# Autodesk Inventor assembly: Assembly
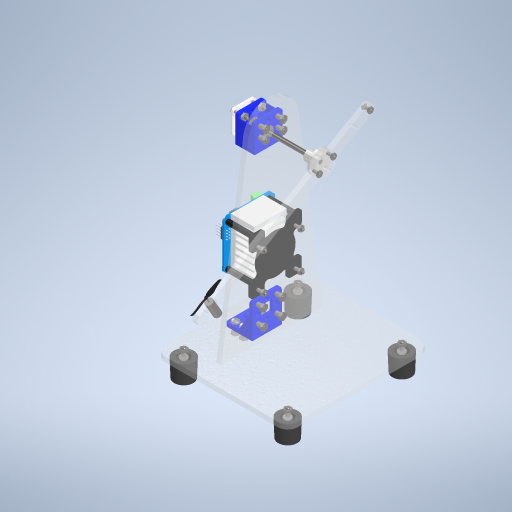
[picture p0: Inventor's stored thumbnail of the model, 512x512]
Saved by Autodesk Inventor 2023.1 (Build 271208000, 208)
## iProperties
Created: 2023-05-07
Part Number: Assembly
Document SubType Name: Assembly
Designer: felip
Author: felip
## Documents named in this file (25)
- C:\Users\felip\OneDrive\UNAL FORE\SEMESTRE 9\TECNICAS DE CONTROL\PROYECTO\PROYECTO-TDC-INVENTOR\Assembly.iam
- C:\Users\felip\OneDrive\UNAL FORE\SEMESTRE 9\TECNICAS DE CONTROL\PROYECTO\PROYECTO-TDC-INVENTOR\base.ipt
- C:\Users\felip\OneDrive\UNAL FORE\SEMESTRE 9\TECNICAS DE CONTROL\PROYECTO\PROYECTO-TDC-INVENTOR\Pata-Goma.ipt
- C:\Users\felip\OneDrive\UNAL FORE\SEMESTRE 9\TECNICAS DE CONTROL\PROYECTO\PROYECTO-TDC-INVENTOR\BaseParal.ipt
- C:\Users\felip\OneDrive\UNAL FORE\SEMESTRE 9\TECNICAS DE CONTROL\PROYECTO\PROYECTO-TDC-INVENTOR\SoporteUnion.ipt
- C:\Users\felip\OneDrive\UNAL FORE\SEMESTRE 9\TECNICAS DE CONTROL\PROYECTO\PROYECTO-TDC-INVENTOR\SoporteEncoder.ipt
- C:\Users\felip\OneDrive\UNAL FORE\SEMESTRE 9\TECNICAS DE CONTROL\PROYECTO\PROYECTO-TDC-INVENTOR\rodamiento.ipt
- C:\Users\felip\OneDrive\UNAL FORE\SEMESTRE 9\TECNICAS DE CONTROL\PROYECTO\PROYECTO-TDC-INVENTOR\topito.ipt
- C:\Users\felip\OneDrive\UNAL FORE\SEMESTRE 9\TECNICAS DE CONTROL\PROYECTO\PROYECTO-TDC-INVENTOR\brida.ipt
- C:\Users\felip\OneDrive\UNAL FORE\SEMESTRE 9\TECNICAS DE CONTROL\PROYECTO\PROYECTO-TDC-INVENTOR\eje.ipt
- C:\Users\felip\OneDrive\UNAL FORE\SEMESTRE 9\TECNICAS DE CONTROL\PROYECTO\PROYECTO-TDC-INVENTOR\brazo.ipt
- C:\Users\felip\OneDrive\UNAL FORE\SEMESTRE 9\TECNICAS DE CONTROL\PROYECTO\PROYECTO-TDC-INVENTOR\motor.ipt
- C:\Users\felip\OneDrive\UNAL FORE\SEMESTRE 9\TECNICAS DE CONTROL\PROYECTO\PROYECTO-TDC-INVENTOR\helice.ipt
- C:\Users\felip\OneDrive\UNAL FORE\SEMESTRE 9\TECNICAS DE CONTROL\PROYECTO\PROYECTO-TDC-INVENTOR\AS5600 v1.ipt
- C:\Users\felip\OneDrive\Documents\Inventor\Content Center Files\R2023\en-US\BS 4183(7)\BS 4183 - M3,5 x 8(2) III.ipt
- C:\Users\felip\OneDrive\Documents\Inventor\Content Center Files\R2023\en-US\BS 4183(4)\BS 4183 - M3,5 x 10(1) III.ipt
- C:\Users\felip\OneDrive\Documents\Inventor\Content Center Files\R2023\en-US\BS 4183(4)\BS 4183 - M2,5 x 10(1) III.ipt
- C:\Users\felip\OneDrive\Documents\Inventor\Content Center Files\R2023\en-US\BS 4183(4)\BS 4183 - M2,5 x 14(1) III.ipt
- C:\Users\felip\OneDrive\Documents\Inventor\Content Center Files\R2023\en-US\BS 4183(4)\BS 4183 - M2,5 x 9(1) III.ipt
- C:\Users\felip\OneDrive\Documents\Inventor\Content Center Files\R2023\en-US\BS 4183(4)\BS 4183 - M2,5 x 7(1) III.ipt
- C:\Users\felip\OneDrive\Documents\Inventor\Content Center Files\R2023\en-US\BS 4183(1)\BS 4183 - M3,5(1).ipt
- C:\Users\felip\OneDrive\Documents\Inventor\Content Center Files\R2023\en-US\BS 4183(1)\BS 4183 - M2,5(1).ipt
- C:\Users\felip\OneDrive\UNAL FORE\SEMESTRE 9\TECNICAS DE CONTROL\PROYECTO\PROYECTO-TDC-INVENTOR\BTS7960 43A HIGH POWER H BRIDGE MODULE.iam
- C:\Users\felip\OneDrive\UNAL FORE\SEMESTRE 9\TECNICAS DE CONTROL\PROYECTO\PROYECTO-TDC-INVENTOR\soporteHBridge.ipt
- C:\Users\felip\OneDrive\Documents\Inventor\Content Center Files\R2023\en-US\BS 4183(4)\BS 4183 - M3 x 7(1) III.ipt
## Components (74 placed, 24 different names)
1. base:1 — Rotational:1, Rotational:2, Rotational:3, Rotational:4, Mate:1, Mate:2, Rotational:5, Rotational:6, Insert:4, Insert:5, Insert:6, Insert:7, Insert:39, Insert:44, Insert:45, Insert:46, Insert:60, Insert:61, Insert:62, Insert:63
2. Pata-Goma:1 — Rotational:1
3. Pata-Goma:2 — Rotational:2
4. Pata-Goma:3 — Rotational:3
5. Pata-Goma:4 — Rotational:4
6. BaseParal:1 — Mate:1, Mate:3, Rotational:7, Rotational:10, Rotational:11, Insert:47, Insert:48, Insert:49, Insert:50, Insert:51, Insert:53, Insert:54, Insert:55, Insert:56, Insert:57, Insert:58, Insert:59, Mate:8, Rotational:20, Rotational:21
7. SoporteUnion:1 — Mate:2, Rotational:5, Rotational:6, Mate:3, Rotational:7, Insert:8, Insert:10, Insert:11, Insert:12, Insert:13, Insert:15, Insert:17, Insert:18
8. SoporteEncoder:1 — Rotational:10, Rotational:11, Insert:1, Insert:2, Rotational:12, Rotational:13, Insert:29, Insert:30, Insert:31, Insert:33, Insert:67, Insert:68
9. rodamiento:1 — Insert:2, Rotational:14
10. rodamiento:2 — Insert:1
11. topito:1 — Rotational:12, Rotational:18
12. topito:2 — Rotational:13, Rotational:19
13. brida:1 — Insert:3, Mate:6, Rotational:15, Rotational:16, Insert:34, Insert:36
14. eje:1 — Rotational:14, Insert:3
15. brazo:1 — Mate:6, Rotational:15, Rotational:16, Flush:1, Tangent:1, Tangent:2, Insert:38, Insert:64, Insert:65, Insert:66
16. motor:1 — Flush:1, Tangent:1, Angle:1, Mate:7, Rotational:17
17. helice:1 — Rotational:17
18. AS5600 v1:1 — Rotational:18, Rotational:19, Insert:25, Insert:28
19. BS 4183 Slotted Pan Head Machine Screw - Metric M3,5 x 8:1 — Insert:4
20. BS 4183 Slotted Pan Head Machine Screw - Metric M3,5 x 8:2 — Insert:5
21. BS 4183 Slotted Pan Head Machine Screw - Metric M3,5 x 8:3 — Insert:6
22. BS 4183 Slotted Pan Head Machine Screw - Metric M3,5 x 8:4 — Insert:7
23. BS 4183 Specification for machine screws and machine screw nuts. Metric series - Metric M3,5 x 10:1 — Insert:8
24. BS 4183 Specification for machine screws and machine screw nuts. Metric series - Metric M3,5 x 10:3 — Insert:10
25. BS 4183 Specification for machine screws and machine screw nuts. Metric series - Metric M3,5 x 10:4 — Insert:11
26. BS 4183 Specification for machine screws and machine screw nuts. Metric series - Metric M3,5 x 10:5 — Insert:12
27. BS 4183 Specification for machine screws and machine screw nuts. Metric series - Metric M3,5 x 10:6 — Insert:13
28. BS 4183 Specification for machine screws and machine screw nuts. Metric series - Metric M3,5 x 10:8 — Insert:15
29. BS 4183 Specification for machine screws and machine screw nuts. Metric series - Metric M3,5 x 10:10 — Insert:17
30. BS 4183 Specification for machine screws and machine screw nuts. Metric series - Metric M3,5 x 10:11 — Insert:18
31. BS 4183 Specification for machine screws and machine screw nuts. Metric series - Metric M2,5 x 10:1
32. BS 4183 Specification for machine screws and machine screw nuts. Metric series - Metric M2,5 x 10:2
33. BS 4183 Specification for machine screws and machine screw nuts. Metric series - Metric M2,5 x 10:3
34. BS 4183 Specification for machine screws and machine screw nuts. Metric series - Metric M2,5 x 10:4
35. BS 4183 Specification for machine screws and machine screw nuts. Metric series - Metric M2,5 x 14:1 — Insert:25
36. BS 4183 Specification for machine screws and machine screw nuts. Metric series - Metric M2,5 x 14:4 — Insert:28
37. BS 4183 Specification for machine screws and machine screw nuts. Metric series - Metric M3,5 x 10:14 — Insert:29
38. BS 4183 Specification for machine screws and machine screw nuts. Metric series - Metric M3,5 x 10:15 — Insert:30
39. BS 4183 Specification for machine screws and machine screw nuts. Metric series - Metric M3,5 x 10:16 — Insert:31
40. BS 4183 Specification for machine screws and machine screw nuts. Metric series - Metric M3,5 x 10:18 — Insert:33
41. BS 4183 Specification for machine screws and machine screw nuts. Metric series - Metric M2,5 x 9:1 — Insert:34
42. BS 4183 Specification for machine screws and machine screw nuts. Metric series - Metric M2,5 x 9:3 — Insert:36
43. BS 4183 Specification for machine screws and machine screw nuts. Metric series - Metric M2,5 x 7:1 — Insert:38
44. BS 4183 - Metric M3,5:1 — Insert:39
45. BS 4183 - Metric M3,5:6 — Insert:44
46. BS 4183 - Metric M3,5:7 — Insert:45
47. BS 4183 - Metric M3,5:8 — Insert:46
48. BS 4183 - Metric M3,5:9 — Insert:47
49. BS 4183 - Metric M3,5:10 — Insert:48
50. BS 4183 - Metric M3,5:11 — Insert:49
51. BS 4183 - Metric M3,5:12 — Insert:50
52. BS 4183 - Metric M3,5:13 — Insert:51
53. BS 4183 - Metric M3,5:15 — Insert:53
54. BS 4183 - Metric M3,5:16 — Insert:54
55. BS 4183 - Metric M3,5:17 — Insert:55
56. BS 4183 - Metric M2,5:1 — Insert:56
57. BS 4183 - Metric M2,5:2 — Insert:57
58. BS 4183 - Metric M2,5:3 — Insert:58
59. BS 4183 - Metric M2,5:4 — Insert:59
60. BS 4183 - Metric M3,5:18 — Insert:60
61. BS 4183 - Metric M3,5:19 — Insert:61
62. BS 4183 - Metric M3,5:20 — Insert:62
63. BS 4183 - Metric M3,5:21 — Insert:63
64. BS 4183 - Metric M2,5:5 — Insert:64
65. BS 4183 - Metric M2,5:6 — Insert:65
66. BS 4183 - Metric M2,5:7 — Insert:66
67. BS 4183 - Metric M3,5:22 — Insert:67
68. BS 4183 - Metric M3,5:23 — Insert:68
69. BTS7960 43A HIGH POWER H BRIDGE MODULE:1 [sub-assembly] — Mate:9, Rotational:22, Rotational:23, Insert:69, Insert:72, Insert:73, Insert:74
70. soporteHBridge:1 — Mate:8, Rotational:20, Rotational:21, Mate:9, Rotational:22, Rotational:23
71. BS 4183 Specification for machine screws and machine screw nuts. Metric series - Metric M3 x 7:1 — Insert:69
72. BS 4183 Specification for machine screws and machine screw nuts. Metric series - Metric M3 x 7:4 — Insert:72
73. BS 4183 Specification for machine screws and machine screw nuts. Metric series - Metric M3 x 7:5 — Insert:73
74. BS 4183 Specification for machine screws and machine screw nuts. Metric series - Metric M3 x 7:6 — Insert:74
## Relationships (85: Insert 53, RevoluteJoint 21, Mate 7, Tangent 2, Flush 1, Angle 1)
- Rotational:1 [RevoluteJoint]: base:1 ↔ Pata-Goma:1
- Rotational:2 [RevoluteJoint]: base:1 ↔ Pata-Goma:2
- Rotational:3 [RevoluteJoint]: base:1 ↔ Pata-Goma:3
- Rotational:4 [RevoluteJoint]: base:1 ↔ Pata-Goma:4
- Mate:1: base:1 ↔ BaseParal:1
- Mate:2: base:1 ↔ SoporteUnion:1
- Rotational:5 [RevoluteJoint]: base:1 ↔ SoporteUnion:1
- Rotational:6 [RevoluteJoint]: base:1 ↔ SoporteUnion:1
- Mate:3: BaseParal:1 ↔ SoporteUnion:1
- Rotational:7 [RevoluteJoint]: BaseParal:1 ↔ SoporteUnion:1
- Rotational:10 [RevoluteJoint]: BaseParal:1 ↔ SoporteEncoder:1
- Rotational:11 [RevoluteJoint]: BaseParal:1 ↔ SoporteEncoder:1
- Insert:1: SoporteEncoder:1 ↔ rodamiento:2
- Insert:2: SoporteEncoder:1 ↔ rodamiento:1
- Rotational:12 [RevoluteJoint]: SoporteEncoder:1 ↔ topito:1
- Rotational:13 [RevoluteJoint]: SoporteEncoder:1 ↔ topito:2
- Rotational:14 [RevoluteJoint]: rodamiento:1 ↔ eje:1
- Insert:3: brida:1 ↔ eje:1
- Mate:6: brida:1 ↔ brazo:1
- Rotational:15 [RevoluteJoint]: brida:1 ↔ brazo:1
- Rotational:16 [RevoluteJoint]: brida:1 ↔ brazo:1
- Flush:1: brazo:1 ↔ motor:1
- Tangent:1: brazo:1 ↔ motor:1
- Angle:1 (0 deg): motor:1
- Tangent:2: brazo:1
- Mate:7 (-15.5 mm): motor:1
- Rotational:17 [RevoluteJoint]: motor:1 ↔ helice:1
- Rotational:18 [RevoluteJoint]: topito:1 ↔ AS5600 v1:1
- Rotational:19 [RevoluteJoint]: topito:2 ↔ AS5600 v1:1
- Insert:4: base:1 ↔ BS 4183 Slotted Pan Head Machine Screw - Metric M3,5 x 8:1
- Insert:5: base:1 ↔ BS 4183 Slotted Pan Head Machine Screw - Metric M3,5 x 8:2
- Insert:6: base:1 ↔ BS 4183 Slotted Pan Head Machine Screw - Metric M3,5 x 8:3
- Insert:7: base:1 ↔ BS 4183 Slotted Pan Head Machine Screw - Metric M3,5 x 8:4
- Insert:8: SoporteUnion:1 ↔ BS 4183 Specification for machine screws and machine screw nuts. Metric series - Metric M3,5 x 10:1
- Insert:10: SoporteUnion:1 ↔ BS 4183 Specification for machine screws and machine screw nuts. Metric series - Metric M3,5 x 10:3
- Insert:11: SoporteUnion:1 ↔ BS 4183 Specification for machine screws and machine screw nuts. Metric series - Metric M3,5 x 10:4
- Insert:12: SoporteUnion:1 ↔ BS 4183 Specification for machine screws and machine screw nuts. Metric series - Metric M3,5 x 10:5
- Insert:13: SoporteUnion:1 ↔ BS 4183 Specification for machine screws and machine screw nuts. Metric series - Metric M3,5 x 10:6
- Insert:15: SoporteUnion:1 ↔ BS 4183 Specification for machine screws and machine screw nuts. Metric series - Metric M3,5 x 10:8
- Insert:17: SoporteUnion:1 ↔ BS 4183 Specification for machine screws and machine screw nuts. Metric series - Metric M3,5 x 10:10
- Insert:18: SoporteUnion:1 ↔ BS 4183 Specification for machine screws and machine screw nuts. Metric series - Metric M3,5 x 10:11
- Insert:25: AS5600 v1:1 ↔ BS 4183 Specification for machine screws and machine screw nuts. Metric series - Metric M2,5 x 14:1
- Insert:28: AS5600 v1:1 ↔ BS 4183 Specification for machine screws and machine screw nuts. Metric series - Metric M2,5 x 14:4
- Insert:29: SoporteEncoder:1 ↔ BS 4183 Specification for machine screws and machine screw nuts. Metric series - Metric M3,5 x 10:14
- Insert:30: SoporteEncoder:1 ↔ BS 4183 Specification for machine screws and machine screw nuts. Metric series - Metric M3,5 x 10:15
- Insert:31: SoporteEncoder:1 ↔ BS 4183 Specification for machine screws and machine screw nuts. Metric series - Metric M3,5 x 10:16
- Insert:33: SoporteEncoder:1 ↔ BS 4183 Specification for machine screws and machine screw nuts. Metric series - Metric M3,5 x 10:18
- Insert:34: brida:1 ↔ BS 4183 Specification for machine screws and machine screw nuts. Metric series - Metric M2,5 x 9:1
- Insert:36: brida:1 ↔ BS 4183 Specification for machine screws and machine screw nuts. Metric series - Metric M2,5 x 9:3
- Insert:38: brazo:1 ↔ BS 4183 Specification for machine screws and machine screw nuts. Metric series - Metric M2,5 x 7:1
- Insert:39: base:1 ↔ BS 4183 - Metric M3,5:1
- Insert:44: base:1 ↔ BS 4183 - Metric M3,5:6
- Insert:45: base:1 ↔ BS 4183 - Metric M3,5:7
- Insert:46: base:1 ↔ BS 4183 - Metric M3,5:8
- Insert:47: BaseParal:1 ↔ BS 4183 - Metric M3,5:9
- Insert:48: BaseParal:1 ↔ BS 4183 - Metric M3,5:10
- Insert:49: BaseParal:1 ↔ BS 4183 - Metric M3,5:11
- Insert:50: BaseParal:1 ↔ BS 4183 - Metric M3,5:12
- Insert:51: BaseParal:1 ↔ BS 4183 - Metric M3,5:13
- Insert:53: BaseParal:1 ↔ BS 4183 - Metric M3,5:15
- Insert:54: BaseParal:1 ↔ BS 4183 - Metric M3,5:16
- Insert:55: BaseParal:1 ↔ BS 4183 - Metric M3,5:17
- Insert:56: BaseParal:1 ↔ BS 4183 - Metric M2,5:1
- Insert:57: BaseParal:1 ↔ BS 4183 - Metric M2,5:2
- Insert:58: BaseParal:1 ↔ BS 4183 - Metric M2,5:3
- Insert:59: BaseParal:1 ↔ BS 4183 - Metric M2,5:4
- Insert:60: base:1 ↔ BS 4183 - Metric M3,5:18
- Insert:61: base:1 ↔ BS 4183 - Metric M3,5:19
- Insert:62: base:1 ↔ BS 4183 - Metric M3,5:20
- Insert:63: base:1 ↔ BS 4183 - Metric M3,5:21
- Insert:64: brazo:1 ↔ BS 4183 - Metric M2,5:5
- Insert:65: brazo:1 ↔ BS 4183 - Metric M2,5:6
- Insert:66: brazo:1 ↔ BS 4183 - Metric M2,5:7
- Insert:67: SoporteEncoder:1 ↔ BS 4183 - Metric M3,5:22
- Insert:68: SoporteEncoder:1 ↔ BS 4183 - Metric M3,5:23
- Mate:8: BaseParal:1 ↔ soporteHBridge:1
- Rotational:20 [RevoluteJoint]: BaseParal:1 ↔ soporteHBridge:1
- Rotational:21 [RevoluteJoint]: BaseParal:1 ↔ soporteHBridge:1
- Mate:9: BTS7960 43A HIGH POWER H BRIDGE MODULE:1 ↔ soporteHBridge:1
- Rotational:22 [RevoluteJoint]: BTS7960 43A HIGH POWER H BRIDGE MODULE:1 ↔ soporteHBridge:1
- Rotational:23 [RevoluteJoint]: BTS7960 43A HIGH POWER H BRIDGE MODULE:1 ↔ soporteHBridge:1
- Insert:69: BTS7960 43A HIGH POWER H BRIDGE MODULE:1 ↔ BS 4183 Specification for machine screws and machine screw nuts. Metric series - Metric M3 x 7:1
- Insert:72: BTS7960 43A HIGH POWER H BRIDGE MODULE:1 ↔ BS 4183 Specification for machine screws and machine screw nuts. Metric series - Metric M3 x 7:4
- Insert:73: BTS7960 43A HIGH POWER H BRIDGE MODULE:1 ↔ BS 4183 Specification for machine screws and machine screw nuts. Metric series - Metric M3 x 7:5
- Insert:74: BTS7960 43A HIGH POWER H BRIDGE MODULE:1 ↔ BS 4183 Specification for machine screws and machine screw nuts. Metric series - Metric M3 x 7:6
